# Autodesk Inventor assembly: 4 Traction, Square_MIR
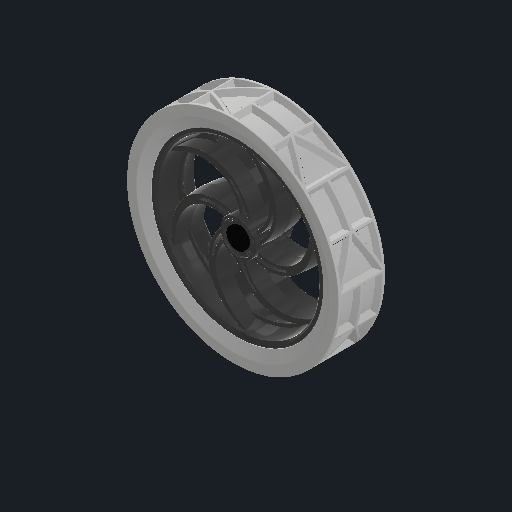
[picture p0: Inventor's stored thumbnail of the model, 512x512]
Saved by Autodesk Inventor 2023 (Build 270158000, 158)
## iProperties
Created: 2022-08-02
Part Number: 4 Traction, Square_MIR
Document SubType Name: Assembly
Designer: Windows Macbook
Author: ylu12
## Documents named in this file (3)
- C:\Users\Windows Macbook\Desktop\VRC-SPIN-UP\Inventor\Motion\Wheels\Traction Wheel\4 Traction, Square_MIR.iam
- C:\Users\Windows Macbook\Desktop\VRC-SPIN-UP\Inventor\Motion\Wheels\Reference Files\4 Traction_MIR.ipt
- C:\Users\Windows Macbook\Desktop\VRC-SPIN-UP\Inventor\Motion\Insert Square_MIR.ipt
## Components (3 placed, 2 different names)
1. 4 Traction_MIR:1 — Mate:12, Mate:11, Flush:6
2. Insert Square_MIR:1 — Angle:2, Mate:28, Symmetry:1
3. Insert Square_MIR:2 — Symmetry:1, Angle:1, Mate:27, Flush:12
## Relationships (9: Mate 5, Angle 2, Flush 1, Symmetry 1)
- Mate:12: 4 Traction_MIR:1
- Mate:11: 4 Traction_MIR:1
- Flush:6: 4 Traction_MIR:1
- Angle:2 (0 deg): Insert Square_MIR:1
- Mate:28: Insert Square_MIR:1
- Symmetry:1: Insert Square_MIR:1 ↔ Insert Square_MIR:2
- Angle:1 (0 deg): Insert Square_MIR:2
- Mate:27: Insert Square_MIR:2
- Flush:12 [Mate] (8.255 mm): Insert Square_MIR:2
## Named parameters: Thickness = 8.255 mm
